# Autodesk Inventor assembly: pcb_shell_ass
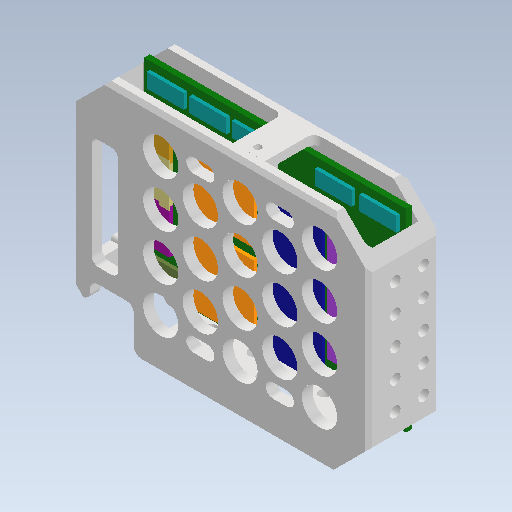
[picture p0: Inventor's stored thumbnail of the model, 512x512]
Saved by Autodesk Inventor 2020 (Build 240168000, 168)
## iProperties
Created: 2019-07-14
Part Number: pcb_shell_ass
Document SubType Name: Assembly
Designer: psrob
Author: psrob
## Documents named in this file (4)
- E:\projects-2\project dog gen2\hardware\pcb_shell_ass.iam
- E:\projects-2\project dog gen2\hardware\ele_3d_2\dog_driver_4.brd.iam
- E:\projects-2\project dog gen2\hardware\pcb_shell_1.ipt
- E:\projects-2\project dog gen2\hardware\pcb_shell_2.ipt
## Components (3 placed, 3 different names)
1. dog_driver_4.brd:1 [sub-assembly] — Flush:1
2. pcb_shell_1:1 — Flush:1, Flush:2
3. pcb_shell_2:1 — Flush:2
## Relationships (2: Flush 2)
- Flush:1: dog_driver_4.brd:1 ↔ pcb_shell_1:1
- Flush:2: pcb_shell_1:1 ↔ pcb_shell_2:1
